# Autodesk Inventor assembly: Assembly1
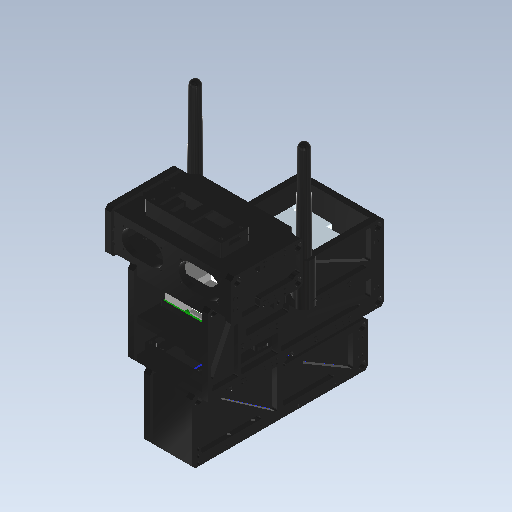
[picture p0: Inventor's stored thumbnail of the model, 512x512]
Saved by Autodesk Inventor 2020 (Build 240168000, 168)
## iProperties
Created: 2021-04-12
Part Number: Assembly1
Document SubType Name: Assembly
Designer: masato
Mass: 658.447 g
Surface Area: 3102.41 cm^2
Volume: 444.276 cm^3
Density: 1.48207 g/cm^3
Author: masato
## Documents named in this file (26)
- C:\Users\Masato\Desktop\最新版\OpenPlatform_ver3_0\上半身\Cockpit\Cockpit.iam
- C:\Users\Masato\Desktop\最新版\OpenPlatform_ver3_0\Ready_Made\Auvidea_J120\Auvidea_J120.ipt
- C:\Users\Masato\Desktop\最新版\OpenPlatform_ver3_0\Ready_Made\Jetson_TX2\Jetson_TX2.ipt
- C:\Users\Masato\Desktop\最新版\OpenPlatform_ver3_0\上半身\Cockpit\Cockpit_vertical_frame_01.ipt
- C:\Users\Masato\Desktop\最新版\OpenPlatform_ver3_0\上半身\Cockpit\Cockpit_vertical_frame_01_MIR.ipt
- C:\Users\Masato\Desktop\最新版\OpenPlatform_ver3_0\上半身\Cockpit\Cockpit_vertical_frame_02.ipt
- C:\Users\Masato\Desktop\最新版\OpenPlatform_ver3_0\Ready_Made\KCD11-A-101011BB.ipt
- C:\Users\Masato\Desktop\最新版\OpenPlatform_ver3_0\上半身\Cockpit\Cockpit_horizontal_frame_01.ipt
- C:\Users\Masato\Desktop\最新版\OpenPlatform_ver3_0\上半身\Cockpit\Antenna_unit.iam
- C:\Users\Masato\Desktop\最新版\OpenPlatform_ver3_0\上半身\Cockpit\Antenna_unit_MIR.iam
- C:\Users\Masato\Desktop\最新版\OpenPlatform_ver3_0\上半身\Cockpit\Cockpit_horizontal_frame_02.ipt
- C:\Users\Masato\Desktop\最新版\OpenPlatform_ver3_0\上半身\Cockpit\Cockpit_vertical_frame_03.ipt
- C:\Users\Masato\Desktop\最新版\OpenPlatform_ver3_0\上半身\Cockpit\Cockpit_vertical_frame_03_MIR.ipt
- C:\Users\Masato\Desktop\最新版\OpenPlatform_ver3_0\上半身\Cockpit\Cockpit_vertical_frame_04.ipt
- C:\Users\Masato\Desktop\最新版\OpenPlatform_ver3_0\上半身\Cockpit\Cockpit_horizontal_frame_03.ipt
- C:\Users\Masato\Desktop\最新版\OpenPlatform_ver3_0\上半身\Cockpit\Cockpit_horizontal_frame_04.ipt
- C:\Users\Masato\Desktop\最新版\OpenPlatform_ver3_0\上半身\Cockpit\Cockpit_vertical_frame_05.ipt
- C:\Users\Masato\Desktop\最新版\OpenPlatform_ver3_0\上半身\Cockpit\Cockpit_vertical_frame_05_MIR.ipt
- C:\Users\Masato\Desktop\最新版\OpenPlatform_ver3_0\上半身\Cockpit\Cockpit_horizontal_frame_05.ipt
- C:\Users\Masato\Desktop\最新版\OpenPlatform_ver3_0\上半身\Cockpit\StartStopSwitch_cover_01.ipt
- C:\Users\Masato\Desktop\最新版\OpenPlatform_ver3_0\上半身\Cockpit\StartStopSwitch_cover_02.ipt
- C:\Users\Masato\Desktop\最新版\OpenPlatform_ver3_0\上半身\Cockpit\Cockpit_vertical_frame_06.ipt
- C:\Users\Masato\Desktop\最新版\OpenPlatform_ver3_0\上半身\Cockpit\Cockpit_vertical_frame_07.ipt
- C:\Users\Masato\Desktop\最新版\OpenPlatform_ver3_0\上半身\Cockpit\Circuit_protection_01.ipt
- C:\Users\Masato\Desktop\最新版\OpenPlatform_ver3_0\Ready_Made\HP-G570-2600S3.ipt
- C:\Users\Masato\Desktop\最新版\OpenPlatform_ver3_0\上半身\Cockpit\Circuit_protection_02.ipt
## Components (26 placed, 25 different names)
1. Auvidea_J120:1 — 挿入:52, 挿入:55, 挿入:90, 挿入:91
2. Jetson_TX2:1 — 挿入:52, 挿入:55
3. KCD11-A-101011BB:1 — メイト:2, メイト:3, メイト:4
4. KCD11-A-101011BB:2 — メイト:13, メイト:14, メイト:15
5. Antenna_unit:1 [sub-assembly] — 挿入:64, 角度:3
6. Antenna_unit_MIR:1 [sub-assembly] — 挿入:95, 角度:10
7. Cockpit_horizontal_frame_01:1 — フラッシュ:1, メイト:8, メイト:9, 挿入:92, 挿入:93
8. Cockpit_horizontal_frame_02:1 — 挿入:67, 挿入:72, 挿入:73, 挿入:87, 挿入:88, 挿入:94
9. Cockpit_horizontal_frame_03:1 — 挿入:74, 挿入:75, メイト:17
10. Cockpit_vertical_frame_01:1 — 挿入:56, 挿入:57, メイト:2, メイト:3, メイト:4, フラッシュ:1, メイト:8, メイト:9, メイト:12, 挿入:64, 角度:3, 挿入:67, 角度:8, 挿入:86, 挿入:94
11. Cockpit_vertical_frame_01_MIR:1 — 挿入:60, 挿入:61, メイト:13, メイト:14, メイト:15, 挿入:95, 角度:10
12. Cockpit_vertical_frame_02:1 — 挿入:56, 挿入:57, 挿入:60, 挿入:61, メイト:10, メイト:11
13. Cockpit_vertical_frame_03:1 — 挿入:68, 挿入:69, 挿入:72, 挿入:74, 挿入:89, 回転:1
14. Cockpit_vertical_frame_03_MIR:1 — 挿入:70, 挿入:71, 挿入:73, 挿入:75, メイト:18
15. Cockpit_vertical_frame_04:1 — 挿入:68, 挿入:69, 挿入:70, 挿入:71, メイト:19
16. Cockpit_horizontal_frame_04:1 — 挿入:98, 角度:11, 挿入:100
17. Cockpit_vertical_frame_05:1 — 挿入:85, 角度:9, 挿入:98, 角度:11, 挿入:99
18. Cockpit_vertical_frame_05_MIR:1 — 挿入:100, 挿入:101
19. Cockpit_horizontal_frame_05:1 — 挿入:99, 挿入:101, 挿入:102, 挿入:103
20. StartStopSwitch_cover_01:1 — 挿入:83, 挿入:84, 挿入:102, 挿入:103
21. StartStopSwitch_cover_02:1 — 挿入:83, 挿入:84
22. Cockpit_vertical_frame_06:1 — 挿入:85, 角度:8, 挿入:86, 角度:9
23. Circuit_protection_01:1 — 挿入:87, 挿入:88
24. HP-G570-2600S3:1 — メイト:17, メイト:18, メイト:19
25. Cockpit_vertical_frame_07:1 — 挿入:89, 回転:1
26. Circuit_protection_02:1 — 挿入:90, 挿入:91, 挿入:92, 挿入:93
## Relationships (56: Insert 35, Mate 14, Angle 5, Flush 1, RevoluteJoint 1)
- 挿入:52 [Insert] (7 mm): Auvidea_J120:1 ↔ Jetson_TX2:1
- 挿入:55 [Insert] (7 mm): Auvidea_J120:1 ↔ Jetson_TX2:1
- 挿入:56 [Insert]: Cockpit_vertical_frame_01:1 ↔ Cockpit_vertical_frame_02:1
- 挿入:57 [Insert]: Cockpit_vertical_frame_01:1 ↔ Cockpit_vertical_frame_02:1
- メイト:2 [Mate]: KCD11-A-101011BB:1 ↔ Cockpit_vertical_frame_01:1
- メイト:3 [Mate] (0.05 mm): KCD11-A-101011BB:1 ↔ Cockpit_vertical_frame_01:1
- メイト:4 [Mate] (0.05 mm): KCD11-A-101011BB:1 ↔ Cockpit_vertical_frame_01:1
- フラッシュ:1 [Flush]: Cockpit_horizontal_frame_01:1 ↔ Cockpit_vertical_frame_01:1
- メイト:8 [Mate] (0.025 mm): Cockpit_horizontal_frame_01:1 ↔ Cockpit_vertical_frame_01:1
- メイト:9 [Mate] (0.025 mm): Cockpit_horizontal_frame_01:1 ↔ Cockpit_vertical_frame_01:1
- 挿入:60 [Insert]: Cockpit_vertical_frame_01_MIR:1 ↔ Cockpit_vertical_frame_02:1
- 挿入:61 [Insert]: Cockpit_vertical_frame_01_MIR:1 ↔ Cockpit_vertical_frame_02:1
- メイト:10 [Mate]: Cockpit_vertical_frame_02:1
- メイト:11 [Mate]: Cockpit_vertical_frame_02:1
- メイト:12 [Mate]: Cockpit_vertical_frame_01:1
- メイト:13 [Mate]: KCD11-A-101011BB:2 ↔ Cockpit_vertical_frame_01_MIR:1
- メイト:14 [Mate] (0.05 mm): KCD11-A-101011BB:2 ↔ Cockpit_vertical_frame_01_MIR:1
- メイト:15 [Mate] (0.05 mm): KCD11-A-101011BB:2 ↔ Cockpit_vertical_frame_01_MIR:1
- 挿入:64 [Insert]: Antenna_unit:1 ↔ Cockpit_vertical_frame_01:1
- 角度:3 [Angle] (0 deg): Antenna_unit:1 ↔ Cockpit_vertical_frame_01:1
- 挿入:67 [Insert]: Cockpit_horizontal_frame_02:1 ↔ Cockpit_vertical_frame_01:1
- 挿入:68 [Insert]: Cockpit_vertical_frame_03:1 ↔ Cockpit_vertical_frame_04:1
- 挿入:69 [Insert]: Cockpit_vertical_frame_03:1 ↔ Cockpit_vertical_frame_04:1
- 挿入:70 [Insert]: Cockpit_vertical_frame_03_MIR:1 ↔ Cockpit_vertical_frame_04:1
- 挿入:71 [Insert]: Cockpit_vertical_frame_03_MIR:1 ↔ Cockpit_vertical_frame_04:1
- 挿入:72 [Insert]: Cockpit_horizontal_frame_02:1 ↔ Cockpit_vertical_frame_03:1
- 挿入:73 [Insert]: Cockpit_horizontal_frame_02:1 ↔ Cockpit_vertical_frame_03_MIR:1
- 挿入:74 [Insert]: Cockpit_horizontal_frame_03:1 ↔ Cockpit_vertical_frame_03:1
- 挿入:75 [Insert]: Cockpit_horizontal_frame_03:1 ↔ Cockpit_vertical_frame_03_MIR:1
- 挿入:83 [Insert] (1.6 mm): StartStopSwitch_cover_01:1 ↔ StartStopSwitch_cover_02:1
- 挿入:84 [Insert] (1.6 mm): StartStopSwitch_cover_01:1 ↔ StartStopSwitch_cover_02:1
- 挿入:85 [Insert]: Cockpit_vertical_frame_05:1 ↔ Cockpit_vertical_frame_06:1
- 角度:8 [Angle] (0 deg): Cockpit_vertical_frame_01:1 ↔ Cockpit_vertical_frame_06:1
- 挿入:86 [Insert]: Cockpit_vertical_frame_01:1 ↔ Cockpit_vertical_frame_06:1
- メイト:17 [Mate]: Cockpit_horizontal_frame_03:1 ↔ HP-G570-2600S3:1
- メイト:18 [Mate]: Cockpit_vertical_frame_03_MIR:1 ↔ HP-G570-2600S3:1
- メイト:19 [Mate]: Cockpit_vertical_frame_04:1 ↔ HP-G570-2600S3:1
- 挿入:87 [Insert]: Cockpit_horizontal_frame_02:1 ↔ Circuit_protection_01:1
- 挿入:88 [Insert]: Cockpit_horizontal_frame_02:1 ↔ Circuit_protection_01:1
- 角度:9 [Angle] (0 deg): Cockpit_vertical_frame_05:1 ↔ Cockpit_vertical_frame_06:1
- 挿入:89 [Insert]: Cockpit_vertical_frame_03:1 ↔ Cockpit_vertical_frame_07:1
- 回転:1 [RevoluteJoint]: Cockpit_vertical_frame_03:1 ↔ Cockpit_vertical_frame_07:1
- 挿入:90 [Insert]: Auvidea_J120:1 ↔ Circuit_protection_02:1
- 挿入:91 [Insert]: Auvidea_J120:1 ↔ Circuit_protection_02:1
- 挿入:92 [Insert]: Cockpit_horizontal_frame_01:1 ↔ Circuit_protection_02:1
- 挿入:93 [Insert]: Cockpit_horizontal_frame_01:1 ↔ Circuit_protection_02:1
- 挿入:94 [Insert]: Cockpit_horizontal_frame_02:1 ↔ Cockpit_vertical_frame_01:1
- 挿入:95 [Insert]: Antenna_unit_MIR:1 ↔ Cockpit_vertical_frame_01_MIR:1
- 角度:10 [Angle] (0 deg): Antenna_unit_MIR:1 ↔ Cockpit_vertical_frame_01_MIR:1
- 挿入:98 [Insert]: Cockpit_horizontal_frame_04:1 ↔ Cockpit_vertical_frame_05:1
- 角度:11 [Angle] (0 deg): Cockpit_horizontal_frame_04:1 ↔ Cockpit_vertical_frame_05:1
- 挿入:99 [Insert]: Cockpit_vertical_frame_05:1 ↔ Cockpit_horizontal_frame_05:1
- 挿入:100 [Insert]: Cockpit_horizontal_frame_04:1 ↔ Cockpit_vertical_frame_05_MIR:1
- 挿入:101 [Insert]: Cockpit_vertical_frame_05_MIR:1 ↔ Cockpit_horizontal_frame_05:1
- 挿入:102 [Insert]: Cockpit_horizontal_frame_05:1 ↔ StartStopSwitch_cover_01:1
- 挿入:103 [Insert]: Cockpit_horizontal_frame_05:1 ↔ StartStopSwitch_cover_01:1
